# Autodesk Inventor assembly: rev2
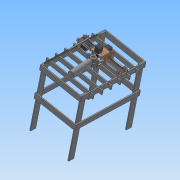
[picture p0: Inventor's stored thumbnail of the model, 180x180]
Saved by Autodesk Inventor 2015 (Build 190159000, 159)
## iProperties
Created: 2014-09-01
Part Number: rev2
Document SubType Name: Assembly
Designer: shohei
Author: shohei
## Documents named in this file (7)
- C:\Users\shohei\Documents\Inventor\PlasmaCNCrev3\Workspaces\Workspace\rev2.iam
- C:\Users\shohei\Documents\Inventor\PlasmaCNCrev3\Workspaces\Workspace\leg.ipt
- C:\Users\shohei\Documents\Inventor\PlasmaCNCrev3\Workspaces\Workspace\leg2.ipt
- C:\Users\shohei\Documents\Inventor\PlasmaCNCrev3\Workspaces\Workspace\leg_zig.ipt
- C:\Users\shohei\Documents\Inventor\PlasmaCNCrev3\Workspaces\Workspace\leg_zag.ipt
- C:\Users\shohei\Documents\Inventor\PlasmaCNCrev3\Workspaces\Workspace\rack_and_pinion.iam
- C:\Users\shohei\Documents\Inventor\PlasmaCNCrev3\slider_rail.ipt
## Components (20 placed, 6 different names)
1. leg:1 — Flush:8, Flush:31, Flush:32, Mate:42, Mate:43, Flush:41
2. leg:2 — Mate:14, Flush:22, Flush:35
3. leg:3 — Flush:6, Mate:3, Mate:12, Mate:13, Mate:15, Flush:27, Flush:28
4. leg:4 — Flush:33, Mate:26, Mate:28
5. leg2:1 — Flush:6, Mate:3, Flush:8, Flush:29, Flush:31, Mate:43
6. leg2:2 — Mate:25, Flush:36, Flush:37, Mate:26, Mate:27, Flush:38
7. leg:8 — Mate:9, Flush:15, Flush:16, Mate:10, Flush:17, Flush:18, Mate:13
8. leg:9 — Mate:29, Flush:39, Flush:40
9. leg2:3 — Mate:9, Flush:15, Flush:16, Mate:12
10. leg2:4 — Mate:10, Flush:17, Flush:18, Mate:29, Flush:39, Flush:40
11. leg_zig:1 — Mate:14, Flush:22, Mate:15, Flush:27, Flush:28, Flush:29, Flush:35, Mate:25, Flush:36, Flush:37, Mate:30, Mate:31, Mate:32
12. leg_zig:2 — Flush:32, Flush:33, Mate:27, Flush:38, Mate:28, Mate:33, Mate:34, Mate:35, Mate:36, Mate:37, Mate:38, Mate:39, Mate:40, Mate:41, Mate:42, Mate:44, Mate:45, Mate:46, Mate:47, Mate:48, Mate:49, Mate:50
13. leg_zag:1 — Mate:30, Mate:31, Mate:32
14. leg_zag:2 — Mate:33, Mate:34, Mate:35
15. leg_zag:3 — Mate:36, Mate:37, Mate:38
16. leg_zag:4 — Mate:39, Mate:40, Mate:41
17. leg_zag:5 — Mate:44, Mate:45, Mate:46
18. leg_zag:6 — Mate:47, Mate:48, Mate:49
19. rack_and_pinion:1 [sub-assembly] — Mate:50, Flush:41
20. slider_rail:1
## Relationships (53: Mate 33, Flush 20)
- Flush:6: leg:3 ↔ leg2:1
- Mate:3: leg:3 ↔ leg2:1
- Flush:8: leg:1 ↔ leg2:1
- Mate:9: leg:8 ↔ leg2:3
- Flush:15: leg:8 ↔ leg2:3
- Flush:16: leg:8 ↔ leg2:3
- Mate:10: leg:8 ↔ leg2:4
- Flush:17: leg:8 ↔ leg2:4
- Flush:18: leg:8 ↔ leg2:4
- Mate:12: leg:3 ↔ leg2:3
- Mate:13: leg:3 ↔ leg:8
- Mate:14: leg:2 ↔ leg_zig:1
- Flush:22: leg:2 ↔ leg_zig:1
- Mate:15: leg:3 ↔ leg_zig:1
- Flush:27: leg:3 ↔ leg_zig:1
- Flush:28: leg:3 ↔ leg_zig:1
- Flush:29: leg2:1 ↔ leg_zig:1
- Flush:31: leg:1 ↔ leg2:1
- Flush:32: leg:1 ↔ leg_zig:2
- Flush:33: leg:4 ↔ leg_zig:2
- Flush:35: leg:2 ↔ leg_zig:1
- Mate:25: leg2:2 ↔ leg_zig:1
- Flush:36: leg2:2 ↔ leg_zig:1
- Flush:37: leg2:2 ↔ leg_zig:1
- Mate:26: leg:4 ↔ leg2:2
- Mate:27: leg2:2 ↔ leg_zig:2
- Flush:38: leg2:2 ↔ leg_zig:2
- Mate:28: leg:4 ↔ leg_zig:2
- Mate:29: leg:9 ↔ leg2:4
- Flush:39: leg:9 ↔ leg2:4
- Flush:40: leg:9 ↔ leg2:4
- Mate:30: leg_zig:1 ↔ leg_zag:1
- Mate:31: leg_zig:1 ↔ leg_zag:1
- Mate:32: leg_zig:1 ↔ leg_zag:1
- Mate:33: leg_zig:2 ↔ leg_zag:2
- Mate:34: leg_zig:2 ↔ leg_zag:2
- Mate:35: leg_zig:2 ↔ leg_zag:2
- Mate:36: leg_zig:2 ↔ leg_zag:3
- Mate:37: leg_zig:2 ↔ leg_zag:3
- Mate:38: leg_zig:2 ↔ leg_zag:3
- Mate:39: leg_zig:2 ↔ leg_zag:4
- Mate:40: leg_zig:2 ↔ leg_zag:4
- Mate:41: leg_zig:2 ↔ leg_zag:4
- Mate:42: leg:1 ↔ leg_zig:2
- Mate:43: leg:1 ↔ leg2:1
- Mate:44: leg_zig:2 ↔ leg_zag:5
- Mate:45: leg_zig:2 ↔ leg_zag:5
- Mate:46: leg_zig:2 ↔ leg_zag:5
- Mate:47: leg_zig:2 ↔ leg_zag:6
- Mate:48: leg_zig:2 ↔ leg_zag:6
- Mate:49: leg_zig:2 ↔ leg_zag:6
- Mate:50: leg_zig:2 ↔ rack_and_pinion:1
- Flush:41: leg:1 ↔ rack_and_pinion:1
